# Autodesk Inventor assembly: Train Assembly Only
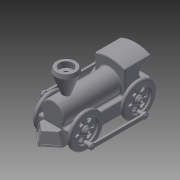
[picture p0: Inventor's stored thumbnail of the model, 180x180]
Saved by Autodesk Inventor 2015 (Build 190159000, 159)
## iProperties
Created: 2018-03-28
Part Number: Train Assembly Only
Document SubType Name: Assembly
Designer: Administrator
Author: Administrator
## Documents named in this file (10)
- L:\IED 9th\8.1a Train\Train Assembly Only.iam
- L:\IED 9th\8.1a Train\Body.ipt
- L:\IED 9th\8.1a Train\Stack.ipt
- L:\IED 9th\8.1a Train\Hitch Magnet.ipt
- L:\IED 9th\8.1a Train\Hitch Peg.ipt
- L:\IED 9th\8.1a Train\Wheel.ipt
- L:\IED 9th\8.1a Train\Axle Peg.ipt
- L:\IED 9th\8.1a Train\Linkage Arm.ipt
- L:\IED 9th\8.1a Train\Linkage Peg.ipt
- L:\IED 9th\8.1a Train\Cow Catcher.ipt
## Components (19 placed, 9 different names)
1. Body:1 — Insert:1, Insert:3, Insert:5, Insert:7, Insert:9, Insert:19, Insert:20, Insert:21, Angle:1
2. Stack:1 — Insert:1
3. Hitch Magnet:1 — Insert:18, Insert:19
4. Hitch Peg:1 — Insert:18
5. Wheel:1 — Insert:6, Insert:7, Insert:17
6. Wheel:2 — Insert:8, Insert:9, Insert:15, Flush:4
7. Wheel:3 — Insert:2, Insert:3, Insert:13
8. Wheel:4 — Insert:4, Insert:5, Insert:11, Angle:1, Flush:4
9. Axle Peg:1 — Insert:2
10. Axle Peg:2 — Insert:4
11. Axle Peg:3 — Insert:6
12. Axle Peg:4 — Insert:8
13. Linkage Arm:1 — Insert:10, Insert:11, Insert:12, Insert:13
14. Linkage Arm:2 — Insert:14, Insert:15, Insert:16, Insert:17
15. Linkage Peg:1 — Insert:16
16. Linkage Peg:2 — Insert:14
17. Linkage Peg:3 — Insert:10
18. Linkage Peg:4 — Insert:12
19. Cow Catcher:1 — Insert:20, Insert:21
## Relationships (23: Insert 21, Angle 1, Flush 1)
- Insert:1: Body:1 ↔ Stack:1
- Insert:2: Wheel:3 ↔ Axle Peg:1
- Insert:3: Body:1 ↔ Wheel:3
- Insert:4: Wheel:4 ↔ Axle Peg:2
- Insert:5: Body:1 ↔ Wheel:4
- Insert:6: Wheel:1 ↔ Axle Peg:3
- Insert:7: Body:1 ↔ Wheel:1
- Insert:8: Wheel:2 ↔ Axle Peg:4
- Insert:9: Body:1 ↔ Wheel:2
- Insert:10: Linkage Arm:1 ↔ Linkage Peg:3
- Insert:11: Wheel:4 ↔ Linkage Arm:1
- Insert:12: Linkage Arm:1 ↔ Linkage Peg:4
- Insert:13: Wheel:3 ↔ Linkage Arm:1
- Insert:14: Linkage Arm:2 ↔ Linkage Peg:2
- Insert:15: Wheel:2 ↔ Linkage Arm:2
- Insert:16: Linkage Arm:2 ↔ Linkage Peg:1
- Insert:17: Wheel:1 ↔ Linkage Arm:2
- Insert:18: Hitch Magnet:1 ↔ Hitch Peg:1
- Insert:19: Body:1 ↔ Hitch Magnet:1
- Insert:20: Body:1 ↔ Cow Catcher:1
- Insert:21: Body:1 ↔ Cow Catcher:1
- Angle:1 (0 deg): Body:1 ↔ Wheel:4
- Flush:4: Wheel:2 ↔ Wheel:4
## Named parameters: crank = 0 deg
